# Autodesk Inventor assembly: CycloidalGear
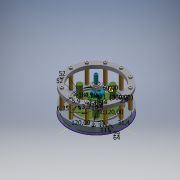
[picture p0: Inventor's stored thumbnail of the model, 180x180]
Saved by Autodesk Inventor 2018.3 (Build 223284000, 284)
## iProperties
Created: 2018-07-20
Part Number: CycloidalGear
Material: Generisch
Document SubType Name: Assembly
Designer: JochenAlt
Author: JochenAlt
## Documents named in this file (6)
- D:\Projects\FlowerPot\CAD\CycloidalGear2\CycloidalGear.iam
- D:\Projects\FlowerPot\CAD\CycloidalGear\MotorShaft.ipt
- C:\Users\JochenAlt\Documents\Inventor\Content Center Files\R2018\de-DE\DIN BEARING(1)\DIN 625 SKF - SKF 623.ipt
- D:\Projects\FlowerPot\CAD\CycloidalGear2\Enclosure.iam
- D:\Projects\FlowerPot\CAD\CycloidalGear2\roulement_61808_2.iam
- D:\Projects\FlowerPot\CAD\CycloidalGear2\Output.iam
## Components (6 placed, 5 different names)
1. DIN 625 SKF SKF 623:1 — Passend:183, Passend:205, Passend:209
2. MotorShaft:8 — Passend:183, Passend:205, Passend:209
3. DIN 625 SKF SKF 623:2
4. Enclosure:1 [sub-assembly] — Passend:218, Passend:219, Passend:223, Passend:224
5. roulement_61808_2:1 [sub-assembly] — Passend:223, Passend:224, Passend:225, Passend:226
6. Output:1 [sub-assembly] — Passend:225, Passend:226
## Relationships (9: Mate 9)
- Passend:183 [Mate]: DIN 625 SKF SKF 623:1 ↔ MotorShaft:8
- Passend:205 [Mate]: DIN 625 SKF SKF 623:1 ↔ MotorShaft:8
- Passend:209 [Mate]: DIN 625 SKF SKF 623:1 ↔ MotorShaft:8
- Passend:218 [Mate]: Enclosure:1
- Passend:219 [Mate]: Enclosure:1
- Passend:223 [Mate]: Enclosure:1 ↔ roulement_61808_2:1
- Passend:224 [Mate]: Enclosure:1 ↔ roulement_61808_2:1
- Passend:225 [Mate]: roulement_61808_2:1 ↔ Output:1
- Passend:226 [Mate]: roulement_61808_2:1 ↔ Output:1
